# Autodesk Inventor assembly: Mould20x20
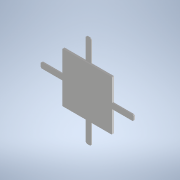
[picture p0: Inventor's stored thumbnail of the model, 180x180]
Saved by Autodesk Inventor 2020.3 (Build 243373010, 373A)
## iProperties
Created: 2020-10-26
Part Number: Mould20x20
Document SubType Name: Assembly
Designer: Naude Conradie
Author: Naude Conradie
## Documents named in this file (4)
- C:\Users\Naude Conradie\Desktop\Repository\Masters-Project\Models\Inventor\Unit Mould\Mould20x20.iam
- C:\Users\Naude Conradie\Desktop\Repository\Masters-Project\Models\Inventor\Unit Mould\MouldBase20x20.ipt
- C:\Users\Naude Conradie\Desktop\Repository\Masters-Project\Models\Inventor\Unit Mould\MouldCell.ipt
- C:\Users\Naude Conradie\Desktop\Repository\Masters-Project\Models\Inventor\Unit Mould\MouldCover20x20.ipt
## Components (6 placed, 3 different names)
1. MouldBase20x20:1 — Mate:1, Mate:2, Mate:3, Mate:4, Mate:5, Mate:6, Mate:7, Mate:8, Mate:9, Mate:10, Mate:11, Mate:12, Flush:1, Flush:2, Mate:13
2. MouldCell:1 — Mate:10, Mate:11, Mate:12
3. MouldCell:2 — Mate:7, Mate:8, Mate:9
4. MouldCell:3 — Mate:4, Mate:5, Mate:6
5. MouldCell:4 — Mate:1, Mate:2, Mate:3
6. MouldCover20x20:1 — Flush:1, Flush:2, Mate:13
## Relationships (15: Mate 13, Flush 2)
- Mate:1: MouldBase20x20:1 ↔ MouldCell:4
- Mate:2: MouldBase20x20:1 ↔ MouldCell:4
- Mate:3: MouldBase20x20:1 ↔ MouldCell:4
- Mate:4: MouldBase20x20:1 ↔ MouldCell:3
- Mate:5: MouldBase20x20:1 ↔ MouldCell:3
- Mate:6: MouldBase20x20:1 ↔ MouldCell:3
- Mate:7: MouldBase20x20:1 ↔ MouldCell:2
- Mate:8: MouldBase20x20:1 ↔ MouldCell:2
- Mate:9: MouldBase20x20:1 ↔ MouldCell:2
- Mate:10: MouldBase20x20:1 ↔ MouldCell:1
- Mate:11: MouldBase20x20:1 ↔ MouldCell:1
- Mate:12: MouldBase20x20:1 ↔ MouldCell:1
- Flush:1: MouldBase20x20:1 ↔ MouldCover20x20:1
- Flush:2: MouldBase20x20:1 ↔ MouldCover20x20:1
- Mate:13: MouldBase20x20:1 ↔ MouldCover20x20:1
